# Autodesk Inventor assembly: CalorimeterAssembly
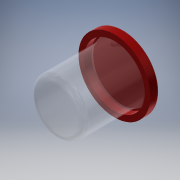
[picture p0: Inventor's stored thumbnail of the model, 180x180]
Saved by Autodesk Inventor 2018.3 (Build 223284000, 284)
## iProperties
Created: 2020-04-09
Part Number: CalorimeterAssembly
Document SubType Name: Assembly
Designer: Ivan
Author: Ivan
## Documents named in this file (4)
- C:\Users\Ivan\Documents\GitHub\Calorimeter\3D Model\CalorimeterAssembly.iam
- C:\Users\Ivan\Documents\GitHub\Calorimeter\3D Model\CalorimeterCap.ipt
- C:\Users\Ivan\Documents\GitHub\Calorimeter\3D Model\Beaker 1L.ipt
- C:\Users\Ivan\Documents\GitHub\Calorimeter\3D Model\IntersectionCube.ipt
## Components (3 placed, 3 different names)
1. CalorimeterCap:1 — Mate:1, Mate:2, Flush:1, Tangent:1
2. Beaker 1L:1 — Mate:1, Mate:2
3. IntersectionCube:1 — Flush:1, Tangent:1, Angle:1
## Relationships (5: Mate 2, Flush 1, Tangent 1, Angle 1)
- Mate:1: CalorimeterCap:1 ↔ Beaker 1L:1
- Mate:2: CalorimeterCap:1 ↔ Beaker 1L:1
- Flush:1: CalorimeterCap:1 ↔ IntersectionCube:1
- Tangent:1: CalorimeterCap:1 ↔ IntersectionCube:1
- Angle:1 (0 deg): IntersectionCube:1
